# Autodesk Inventor assembly: 01001 ASY GBK wall shield Center 10
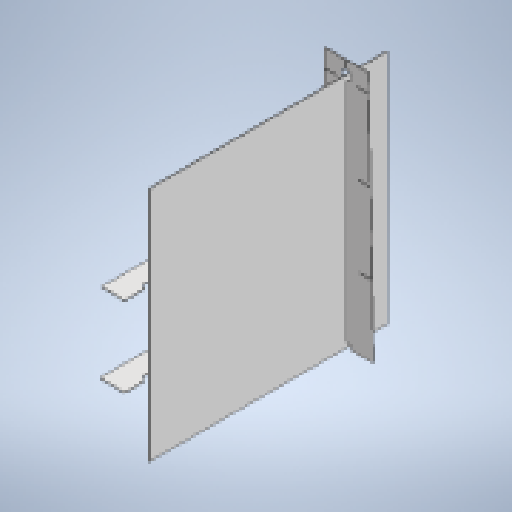
[picture p0: Inventor's stored thumbnail of the model, 512x512]
Saved by Autodesk Inventor 2026 (Build 300175000, 175)
## iProperties
Created: 2026-05-19
Part Number: 01001 ASY GBK wall shield Center 10
Document SubType Name: Assembly
Designer: pokla
Author: admin
## Documents named in this file (5)
- C:\Users\pokla\Documents\Inventor\GBK-Gubkinskiy\01001 ASY GBK wall shield Center 10.iam
- C:\Users\pokla\Documents\Inventor\GBK-Gubkinskiy\01011 GBK Center rib 3.ipt
- C:\Users\pokla\Documents\Inventor\GBK-Gubkinskiy\01013 GBK stringer C7.ipt
- C:\Users\pokla\Documents\Inventor\GBK-Gubkinskiy\010.7 GBK shield.ipt
- C:\Users\pokla\Documents\Inventor\GBK-Gubkinskiy\01014 GBK stringer C8.ipt
## Components (5 placed, 4 different names)
1. 01011 GBK Center rib 3:1 — Совмещение:5, Заподлицо:5, Заподлицо:4, Заподлицо:7, Жесткий:1, Жесткий:2
2. 01013 GBK stringer C7:1 — Жесткий:1
3. 010.7 GBK shield:1 — Совмещение:1, Заподлицо:1, Совмещение:2, Совмещение:5, Заподлицо:5, Совмещение:4, Заподлицо:6, Заподлицо:7
4. 01011 GBK Center rib 3:2 — Совмещение:4, Заподлицо:4, Заподлицо:6
5. 01014 GBK stringer C8:1 — Жесткий:2
## Relationships (11: Flush 5, Mate 4, WeldJoint 2)
- Совмещение:1 [Mate]: 010.7 GBK shield:1
- Заподлицо:1 [Flush]: 010.7 GBK shield:1
- Совмещение:2 [Mate]: 010.7 GBK shield:1
- Совмещение:5 [Mate]: 01011 GBK Center rib 3:1 ↔ 010.7 GBK shield:1
- Заподлицо:5 [Flush] (250 mm): 01011 GBK Center rib 3:1 ↔ 010.7 GBK shield:1
- Совмещение:4 [Mate]: 010.7 GBK shield:1 ↔ 01011 GBK Center rib 3:2
- Заподлицо:4 [Flush]: 01011 GBK Center rib 3:1 ↔ 01011 GBK Center rib 3:2
- Заподлицо:6 [Flush]: 010.7 GBK shield:1 ↔ 01011 GBK Center rib 3:2
- Заподлицо:7 [Flush]: 01011 GBK Center rib 3:1 ↔ 010.7 GBK shield:1
- Жесткий:1 [WeldJoint] (4 mm): 01011 GBK Center rib 3:1 ↔ 01013 GBK stringer C7:1
- Жесткий:2 [WeldJoint] (4 mm): 01011 GBK Center rib 3:1 ↔ 01014 GBK stringer C8:1
